# Autodesk Inventor assembly: QUAT HUT CAO AP
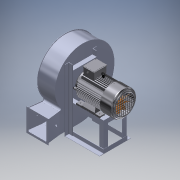
[picture p0: Inventor's stored thumbnail of the model, 180x180]
Saved by Autodesk Inventor 2017 (Build 210142000, 142)
## iProperties
Created: 2013-02-22
Part Number: QUAT HUT CAO AP
Document SubType Name: Assembly
Designer: XuZhiqing
Sending System: SolidWorks 2013
Last Author: Usr01
Last Saved: 2013-03-04
Author: XuZhiqing
## Documents named in this file (6)
- C:\Users\XuZhiqing\Desktop\Project01-CFD_the_sys\CAD-IPT\compressor\QUAT HUT CAO AP.iam
- C:\Users\XuZhiqing\Desktop\Project01-CFD_the_sys\CAD-IPT\compressor\QUAT HUT.iam
- C:\Users\XuZhiqing\Desktop\Project01-CFD_the_sys\CAD-IPT\compressor\CANH.iam
- C:\Users\XuZhiqing\Desktop\Project01-CFD_the_sys\CAD-IPT\compressor\MAT TROI.iam
- C:\Users\XuZhiqing\Desktop\Project01-CFD_the_sys\CAD-IPT\compressor\DAU GIAM AP.iam
- C:\Users\XuZhiqing\Desktop\Project01-CFD_the_sys\CAD-IPT\compressor\User Library-Motor_1LG0186_.ipt
## Components (5 placed, 5 different names)
1. QUAT HUT:1 [sub-assembly] — Flush:1
2. CANH:1 [sub-assembly]
3. Assem2^QUAT HUT CAO AP:1 [sub-assembly] — Flush:1
4. DAU GIAM AP:1 [sub-assembly]
5. User Library-Motor_1LG0186_:1
## Relationships (1: Flush 1)
- Flush:1: QUAT HUT:1 ↔ Assem2^QUAT HUT CAO AP:1
